# Autodesk Inventor assembly: Assembly3
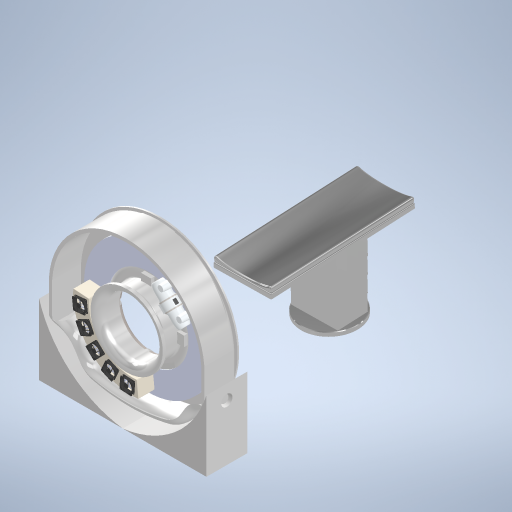
[picture p0: Inventor's stored thumbnail of the model, 512x512]
Saved by Autodesk Inventor 2024 (Build 280153020, 153B)
## iProperties
Created: 2025-04-16
Part Number: Assembly3
Document SubType Name: Assembly
Designer: LENOVO
Author: LENOVO
## Documents named in this file (7)
- C:\Users\LENOVO\OneDrive\Desktop\Assembly3.iam
- C:\Users\LENOVO\OneDrive\Desktop\mov.ct 1 (1).ipt
- C:\Users\LENOVO\OneDrive\Desktop\xray tube (1)\xray tube (1).ipt
- C:\Users\LENOVO\OneDrive\Desktop\ct gantry plate (1)\ct gantry plate (1).ipt
- C:\Users\LENOVO\OneDrive\Desktop\detector assemb (1)\detector assemb (1).ipt
- C:\Users\LENOVO\OneDrive\Desktop\CT Scanner stand1.ipt
- C:\Users\LENOVO\OneDrive\Desktop\stand111.ipt
## Components (6 placed, 6 different names)
1. mov.ct 1 (1):1 — Rotational:1, Rigid:2
2. xray tube (1):1 — Rotational:2, Rotational:3
3. ct gantry plate (1):1 — Rotational:1, Rotational:2, Rotational:3, Rigid:1
4. detector assemb (1):1 — Rigid:1
5. CT Scanner stand1:1
6. stand111:1 — Rigid:2
## Relationships (5: RevoluteJoint 3, WeldJoint 2)
- Rotational:1 [RevoluteJoint]: mov.ct 1 (1):1 ↔ ct gantry plate (1):1
- Rotational:2 [RevoluteJoint]: xray tube (1):1 ↔ ct gantry plate (1):1
- Rotational:3 [RevoluteJoint]: xray tube (1):1 ↔ ct gantry plate (1):1
- Rigid:1 [WeldJoint]: ct gantry plate (1):1 ↔ detector assemb (1):1
- Rigid:2 [WeldJoint]: mov.ct 1 (1):1 ↔ stand111:1
